# Autodesk Inventor assembly: 000.005.002 - Плечо СБ
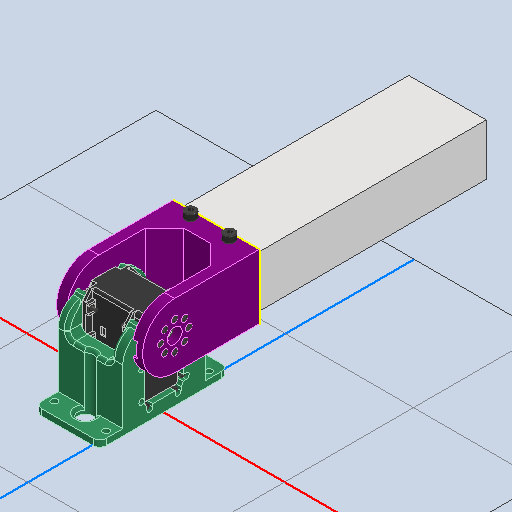
[picture p0: Inventor's stored thumbnail of the model, 512x512]
Saved by Autodesk Inventor 2022 (Build 260153000, 153)
## iProperties
Created: 2022-11-17
Part Number: 000.005.002 - Плечо СБ
Document SubType Name: Assembly
Designer: Petrov Ivan
Author: Petrov Ivan
## Documents named in this file (13)
- C:\Users\Ivan Petrov\Documents\GitHub\OmniBot\design\000.005.002 - Плечо СБ.iam
- C:\Users\Ivan Petrov\Documents\GitHub\OmniBot\design\000.005.002.001 - Основание.ipt
- C:\Users\Ivan Petrov\Documents\GitHub\OmniBot\design\standart_components\dynamixels\mx-106\MX106T.iam
- C:\Users\Ivan Petrov\Documents\GitHub\OmniBot\design\Content Center Files\R2022\ru-RU\BS EN 24035\ISO 4035 - M2,5BS EN.ipt
- C:\Users\Ivan Petrov\Documents\GitHub\OmniBot\design\000.005.002.002 - Качалка.ipt
- C:\Users\Ivan Petrov\Documents\GitHub\OmniBot\design\Content Center Files\R2022\ru-RU\ISO 4762(1)\DIN EN ISO 4762 - M2,5 x 8.ipt
- C:\Users\Ivan Petrov\Documents\GitHub\OmniBot\design\Content Center Files\R2022\ru-RU\SKF 2RS1 -  with two seals\SKF 2RS1608-2RS1.ipt
- C:\Users\Ivan Petrov\Documents\GitHub\OmniBot\design\000.005.002.003 - Втулка.ipt
- C:\Users\Ivan Petrov\Documents\GitHub\OmniBot\design\Content Center Files\R2022\ru-RU\ISO 4762(1)\DIN EN ISO 4762 - M2,5 x 12.ipt
- C:\Users\Ivan Petrov\Documents\GitHub\OmniBot\design\Content Center Files\R2022\ru-RU\BS EN 24032\ISO 4032 - M5BS EN.ipt
- C:\Users\Ivan Petrov\Documents\GitHub\OmniBot\design\Content Center Files\R2022\ru-RU\ISO 4762(1)\DIN EN ISO 4762 - M5 x 20.ipt
- C:\Users\Ivan Petrov\Documents\GitHub\OmniBot\design\Content Center Files\R2022\ru-RU\ISO 4762(1)\DIN EN ISO 4762 - M2,5 x 10.ipt
- C:\Users\Ivan Petrov\Documents\GitHub\OmniBot\design\000.005.002.004 - Рычаг.ipt
## Components (47 placed, 12 different names)
1. 000.005.002.001 - Основание:1 — Совмещение:1, Совмещение:2, Заподлицо:1, Вставка:9, Вставка:10, Вставка:11, Вставка:12, Вставка:13, Вставка:14, Вставка:15, Вставка:16, Вставка:17, Вставка:18, Вставка:19, Вставка:20, Вставка:21, Вставка:22, Вставка:23, Вставка:24
2. MX106T:1 [sub-assembly] — Совмещение:1, Совмещение:2, Заподлицо:1, Вставка:1, Вставка:2, Вставка:3, Вставка:4, Вставка:5, Вставка:6, Вставка:7, Вставка:8, Совмещение:3, Совмещение:4, Совмещение:5, Совмещение:6, Совмещение:7, Совмещение:10
3. 000.005.002.002 - Качалка:1 — Совмещение:3, Совмещение:4, Совмещение:5, Вставка:25, Вставка:26, Вставка:27, Вставка:28, Вставка:29, Вставка:30, Вставка:31, Вставка:32, Совмещение:11, Совмещение:12, Совмещение:13, Вставка:34, Вставка:35, Вставка:36, Вставка:37, Вставка:38, Вставка:39, Вставка:40, Вставка:41
4. SKF 2RS1, с двумя уплотнениями SKF 2RS1608-2RS1:1 — Совмещение:6, Совмещение:7, Совмещение:9
5. 000.005.002.003 - Втулка:1 — Совмещение:9, Совмещение:10, Вставка:33
6. DIN EN ISO 4762 M2,5 x 12:1 — Вставка:33
7. 000.005.002.004 - Рычаг:1 — Совмещение:11, Совмещение:12, Совмещение:13
8. BS EN 24032 - метрическая M5:1 — Вставка:34
9. BS EN 24032 - метрическая M5:2 — Вставка:35
10. BS EN 24032 - метрическая M5:3 — Вставка:36
11. BS EN 24032 - метрическая M5:4 — Вставка:37
12. DIN EN ISO 4762 M5 x 20:1 — Вставка:38
13. DIN EN ISO 4762 M5 x 20:2 — Вставка:39
14. DIN EN ISO 4762 M5 x 20:3 — Вставка:40
15. DIN EN ISO 4762 M5 x 20:4 — Вставка:41
16. DIN EN ISO 4762 M2,5 x 8:1 — Вставка:25
17. DIN EN ISO 4762 M2,5 x 8:2 — Вставка:26
18. DIN EN ISO 4762 M2,5 x 8:3 — Вставка:27
19. DIN EN ISO 4762 M2,5 x 8:4 — Вставка:28
20. DIN EN ISO 4762 M2,5 x 8:5 — Вставка:29
21. DIN EN ISO 4762 M2,5 x 8:6 — Вставка:30
22. DIN EN ISO 4762 M2,5 x 8:7 — Вставка:31
23. DIN EN ISO 4762 M2,5 x 8:8 — Вставка:32
24. BS EN 24035 - метрическая M2,5:1 — Вставка:1
25. BS EN 24035 - метрическая M2,5:2 — Вставка:2
26. BS EN 24035 - метрическая M2,5:3 — Вставка:3
27. BS EN 24035 - метрическая M2,5:4 — Вставка:4
28. BS EN 24035 - метрическая M2,5:5 — Вставка:5
29. BS EN 24035 - метрическая M2,5:6 — Вставка:6
30. BS EN 24035 - метрическая M2,5:7 — Вставка:7
31. BS EN 24035 - метрическая M2,5:8 — Вставка:8
32. DIN EN ISO 4762 M2,5 x 10:1 — Вставка:9
33. DIN EN ISO 4762 M2,5 x 10:2 — Вставка:10
34. DIN EN ISO 4762 M2,5 x 10:3 — Вставка:11
35. DIN EN ISO 4762 M2,5 x 10:4 — Вставка:12
36. DIN EN ISO 4762 M2,5 x 10:5 — Вставка:13
37. DIN EN ISO 4762 M2,5 x 10:6 — Вставка:14
38. DIN EN ISO 4762 M2,5 x 10:7 — Вставка:15
39. DIN EN ISO 4762 M2,5 x 10:8 — Вставка:16
40. DIN EN ISO 4762 M2,5 x 10:9 — Вставка:17
41. DIN EN ISO 4762 M2,5 x 10:10 — Вставка:18
42. DIN EN ISO 4762 M2,5 x 10:11 — Вставка:19
43. DIN EN ISO 4762 M2,5 x 10:12 — Вставка:20
44. DIN EN ISO 4762 M2,5 x 10:13 — Вставка:21
45. DIN EN ISO 4762 M2,5 x 10:14 — Вставка:22
46. DIN EN ISO 4762 M2,5 x 10:15 — Вставка:23
47. DIN EN ISO 4762 M2,5 x 10:16 — Вставка:24
## Relationships (54: Insert 41, Mate 12, Flush 1)
- Совмещение:1 [Mate]: 000.005.002.001 - Основание:1 ↔ MX106T:1
- Совмещение:2 [Mate]: 000.005.002.001 - Основание:1 ↔ MX106T:1
- Заподлицо:1 [Flush] (-0.25 mm): 000.005.002.001 - Основание:1 ↔ MX106T:1
- Вставка:1 [Insert]: MX106T:1 ↔ BS EN 24035 - метрическая M2,5:1
- Вставка:2 [Insert]: MX106T:1 ↔ BS EN 24035 - метрическая M2,5:2
- Вставка:3 [Insert]: MX106T:1 ↔ BS EN 24035 - метрическая M2,5:3
- Вставка:4 [Insert]: MX106T:1 ↔ BS EN 24035 - метрическая M2,5:4
- Вставка:5 [Insert]: MX106T:1 ↔ BS EN 24035 - метрическая M2,5:5
- Вставка:6 [Insert]: MX106T:1 ↔ BS EN 24035 - метрическая M2,5:6
- Вставка:7 [Insert]: MX106T:1 ↔ BS EN 24035 - метрическая M2,5:7
- Вставка:8 [Insert]: MX106T:1 ↔ BS EN 24035 - метрическая M2,5:8
- Вставка:9 [Insert]: 000.005.002.001 - Основание:1 ↔ DIN EN ISO 4762 M2,5 x 10:1
- Вставка:10 [Insert]: 000.005.002.001 - Основание:1 ↔ DIN EN ISO 4762 M2,5 x 10:2
- Вставка:11 [Insert]: 000.005.002.001 - Основание:1 ↔ DIN EN ISO 4762 M2,5 x 10:3
- Вставка:12 [Insert]: 000.005.002.001 - Основание:1 ↔ DIN EN ISO 4762 M2,5 x 10:4
- Вставка:13 [Insert]: 000.005.002.001 - Основание:1 ↔ DIN EN ISO 4762 M2,5 x 10:5
- Вставка:14 [Insert]: 000.005.002.001 - Основание:1 ↔ DIN EN ISO 4762 M2,5 x 10:6
- Вставка:15 [Insert]: 000.005.002.001 - Основание:1 ↔ DIN EN ISO 4762 M2,5 x 10:7
- Вставка:16 [Insert]: 000.005.002.001 - Основание:1 ↔ DIN EN ISO 4762 M2,5 x 10:8
- Вставка:17 [Insert]: 000.005.002.001 - Основание:1 ↔ DIN EN ISO 4762 M2,5 x 10:9
- Вставка:18 [Insert]: 000.005.002.001 - Основание:1 ↔ DIN EN ISO 4762 M2,5 x 10:10
- Вставка:19 [Insert]: 000.005.002.001 - Основание:1 ↔ DIN EN ISO 4762 M2,5 x 10:11
- Вставка:20 [Insert]: 000.005.002.001 - Основание:1 ↔ DIN EN ISO 4762 M2,5 x 10:12
- Вставка:21 [Insert]: 000.005.002.001 - Основание:1 ↔ DIN EN ISO 4762 M2,5 x 10:13
- Вставка:22 [Insert]: 000.005.002.001 - Основание:1 ↔ DIN EN ISO 4762 M2,5 x 10:14
- Вставка:23 [Insert]: 000.005.002.001 - Основание:1 ↔ DIN EN ISO 4762 M2,5 x 10:15
- Вставка:24 [Insert]: 000.005.002.001 - Основание:1 ↔ DIN EN ISO 4762 M2,5 x 10:16
- Совмещение:3 [Mate] (0.05 mm): MX106T:1 ↔ 000.005.002.002 - Качалка:1
- Совмещение:4 [Mate]: MX106T:1 ↔ 000.005.002.002 - Качалка:1
- Совмещение:5 [Mate]: MX106T:1 ↔ 000.005.002.002 - Качалка:1
- Вставка:25 [Insert]: 000.005.002.002 - Качалка:1 ↔ DIN EN ISO 4762 M2,5 x 8:1
- Вставка:26 [Insert]: 000.005.002.002 - Качалка:1 ↔ DIN EN ISO 4762 M2,5 x 8:2
- Вставка:27 [Insert]: 000.005.002.002 - Качалка:1 ↔ DIN EN ISO 4762 M2,5 x 8:3
- Вставка:28 [Insert]: 000.005.002.002 - Качалка:1 ↔ DIN EN ISO 4762 M2,5 x 8:4
- Вставка:29 [Insert]: 000.005.002.002 - Качалка:1 ↔ DIN EN ISO 4762 M2,5 x 8:5
- Вставка:30 [Insert]: 000.005.002.002 - Качалка:1 ↔ DIN EN ISO 4762 M2,5 x 8:6
- Вставка:31 [Insert]: 000.005.002.002 - Качалка:1 ↔ DIN EN ISO 4762 M2,5 x 8:7
- Вставка:32 [Insert]: 000.005.002.002 - Качалка:1 ↔ DIN EN ISO 4762 M2,5 x 8:8
- Совмещение:6 [Mate]: MX106T:1 ↔ SKF 2RS1, с двумя уплотнениями SKF 2RS1608-2RS1:1
- Совмещение:7 [Mate] (0.5 mm): MX106T:1 ↔ SKF 2RS1, с двумя уплотнениями SKF 2RS1608-2RS1:1
- Совмещение:9 [Mate]: SKF 2RS1, с двумя уплотнениями SKF 2RS1608-2RS1:1 ↔ 000.005.002.003 - Втулка:1
- Совмещение:10 [Mate]: MX106T:1 ↔ 000.005.002.003 - Втулка:1
- Вставка:33 [Insert]: 000.005.002.003 - Втулка:1 ↔ DIN EN ISO 4762 M2,5 x 12:1
- Совмещение:11 [Mate]: 000.005.002.002 - Качалка:1 ↔ 000.005.002.004 - Рычаг:1
- Совмещение:12 [Mate] (0.25 mm): 000.005.002.002 - Качалка:1 ↔ 000.005.002.004 - Рычаг:1
- Совмещение:13 [Mate] (0.25 mm): 000.005.002.002 - Качалка:1 ↔ 000.005.002.004 - Рычаг:1
- Вставка:34 [Insert]: 000.005.002.002 - Качалка:1 ↔ BS EN 24032 - метрическая M5:1
- Вставка:35 [Insert]: 000.005.002.002 - Качалка:1 ↔ BS EN 24032 - метрическая M5:2
- Вставка:36 [Insert]: 000.005.002.002 - Качалка:1 ↔ BS EN 24032 - метрическая M5:3
- Вставка:37 [Insert]: 000.005.002.002 - Качалка:1 ↔ BS EN 24032 - метрическая M5:4
- Вставка:38 [Insert]: 000.005.002.002 - Качалка:1 ↔ DIN EN ISO 4762 M5 x 20:1
- Вставка:39 [Insert]: 000.005.002.002 - Качалка:1 ↔ DIN EN ISO 4762 M5 x 20:2
- Вставка:40 [Insert]: 000.005.002.002 - Качалка:1 ↔ DIN EN ISO 4762 M5 x 20:3
- Вставка:41 [Insert]: 000.005.002.002 - Качалка:1 ↔ DIN EN ISO 4762 M5 x 20:4
